# Autodesk Inventor assembly: Top layer
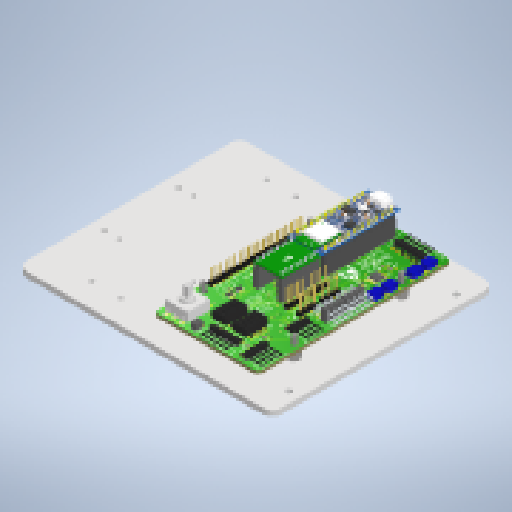
[picture p0: Inventor's stored thumbnail of the model, 512x512]
Saved by Autodesk Inventor 2025.1 (Build 291241000, 241)
## iProperties
Created: 2024-10-04
Part Number: Top layer
Document SubType Name: Assembly
Designer: bw1293
Author: bw1293
## Documents named in this file (4)
- C:\Users\benja\OneDrive\Documents\PlatformIO\Projects\241025-214150-nano33ble\GEOFF-2.0\CAD\Top layer.iam
- C:\Users\benja\OneDrive\Documents\PlatformIO\Projects\241025-214150-nano33ble\GEOFF-2.0\CAD\ARB Board CAD model.ipt
- C:\Users\benja\OneDrive\Documents\PlatformIO\Projects\241025-214150-nano33ble\GEOFF-2.0\CAD\M2.5 Hex Spacer 5mm.ipt
- C:\Users\benja\OneDrive\Documents\PlatformIO\Projects\241025-214150-nano33ble\GEOFF-2.0\CAD\Top base 2.ipt
## Components (6 placed, 3 different names)
1. ARB Board CAD model:1 — Insert:1, Insert:2, Insert:4
2. M2.5 Hex Spacer 5mm:1 — Insert:4, Insert:5
3. M2.5 Hex Spacer 5mm:2 — Insert:7
4. M2.5 Hex Spacer 5mm:3 — Insert:2, Insert:8
5. M2.5 Hex Spacer 5mm:4 — Insert:1, Insert:6
6. Top base 2:1 — Insert:5, Insert:6, Insert:7, Insert:8
## Relationships (7: Insert 7)
- Insert:1: ARB Board CAD model:1 ↔ M2.5 Hex Spacer 5mm:4
- Insert:2: ARB Board CAD model:1 ↔ M2.5 Hex Spacer 5mm:3
- Insert:4: ARB Board CAD model:1 ↔ M2.5 Hex Spacer 5mm:1
- Insert:5: M2.5 Hex Spacer 5mm:1 ↔ Top base 2:1
- Insert:6: M2.5 Hex Spacer 5mm:4 ↔ Top base 2:1
- Insert:7: M2.5 Hex Spacer 5mm:2 ↔ Top base 2:1
- Insert:8: M2.5 Hex Spacer 5mm:3 ↔ Top base 2:1
